# Autodesk Inventor assembly: Assembly2
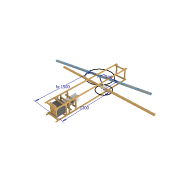
[picture p0: Inventor's stored thumbnail of the model, 180x180]
Saved by Autodesk Inventor 2020 (Build 240168000, 168)
## iProperties
Created: 2022-05-05
Part Number: Assembly2
Document SubType Name: Assembly
Designer: leo
Author: leo
## Documents named in this file (7)
- C:\Users\leo.DESKTOP-592E5E6\Documents\GitHub\TallerDix2022\cad\Inventor\Assembly2.iam
- C:\Users\leo.DESKTOP-592E5E6\Documents\GitHub\TallerDix2022\cad\Inventor\Base listones.ipt
- C:\Users\leo.DESKTOP-592E5E6\Documents\GitHub\TallerDix2022\cad\Inventor\adocreto.ipt
- C:\Users\leo.DESKTOP-592E5E6\Documents\GitHub\TallerDix2022\cad\Inventor\Caja motriz BASE.iam
- C:\Users\leo.DESKTOP-592E5E6\Documents\GitHub\TallerDix2022\cad\Inventor\pieza.ipt
- C:\Users\leo.DESKTOP-592E5E6\Documents\GitHub\TallerDix2022\cad\Inventor\parte móvil.iam
- C:\Users\leo.DESKTOP-592E5E6\Documents\GitHub\TallerDix2022\cad\Inventor\esquema.ipt
## Components (6 placed, 6 different names)
1. Base listones:1
2. adocreto:1 — Flush:1, Flush:2
3. Caja motriz BASE:1 [sub-assembly] — Flush:3, Mate:4
4. parte móvil:1 [sub-assembly] — Mate:2, Mate:4, Rotation:5
5. pieza:1 — Mate:5, Rotation:5
6. esquema:1 — Flush:4, Flush:5, Flush:6, Mate:7, Mate:8
## Relationships (18: Flush 6, Mate 5, RelateRotation 5, Angle 2)
- Flush:1: adocreto:1
- Flush:2: adocreto:1
- Flush:3: Caja motriz BASE:1
- Mate:2: parte móvil:1
- Mate:4: Caja motriz BASE:1 ↔ parte móvil:1
- Mate:5: pieza:1
- Flush:4: esquema:1
- Flush:5: esquema:1
- Flush:6: esquema:1
- Mate:7: esquema:1
- Angle:1 (0 deg)
- Mate:8: esquema:1
- Angle:2 (0 deg)
- Rotation:1 [RelateRotation] (2 ul)
- Rotation:2 [RelateRotation] (2 ul)
- Rotation:3 [RelateRotation] (3 ul)
- Rotation:4 [RelateRotation] (0.5 ul)
- Rotation:5 [RelateRotation] (0.3333 ul): parte móvil:1 ↔ pieza:1
